# Autodesk Inventor assembly: Clamp Assembly
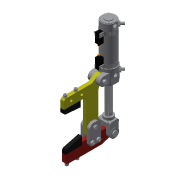
[picture p0: Inventor's stored thumbnail of the model, 180x180]
Saved by Autodesk Inventor 2020.1 (Build 241239000, 239)
## iProperties
Created: 2019-08-27
Part Number: Clamp Assembly
Document SubType Name: Assembly
Designer: thom_tremblay
Author: thom_tremblay
## Documents named in this file (5)
- C:\Users\thomastremblay\Desktop\Inventor ACP Data\Assemblies\Clamp Assembly.iam
- C:\Users\thomastremblay\Desktop\Inventor ACP Data\Assemblies\PH-000-001.iam
- C:\Users\thomastremblay\Desktop\Inventor ACP Data\Assemblies\PH-000-002.iam
- C:\Users\thomastremblay\Desktop\Inventor ACP Data\Assemblies\210-103b.iam
- C:\Users\thomastremblay\Desktop\Inventor ACP Data\Assemblies\210-110b.IAM
## Components (4 placed, 4 different names)
1. PH-000-002:1 [sub-assembly] — Actuator stroke
2. PH-000-001:1 [sub-assembly] — Actuator stroke
3. 210-103b:1 [sub-assembly]
4. 210-110b:1 [sub-assembly]
## Relationships (5: Insert 3, Mate 2)
- [Mate]: PH-000-002:1 ↔ PH-000-001:1
- [Insert]: PH-000-001:1 ↔ 210-103b:1
- [Insert]: 210-103b:1 ↔ 210-110b:1
- [Mate]: PH-000-002:1 ↔ 210-110b:1
- Actuator stroke [Insert] (95.504 mm): PH-000-002:1 ↔ PH-000-001:1
